# Autodesk Inventor assembly: spur_gear_m0.8-18.4
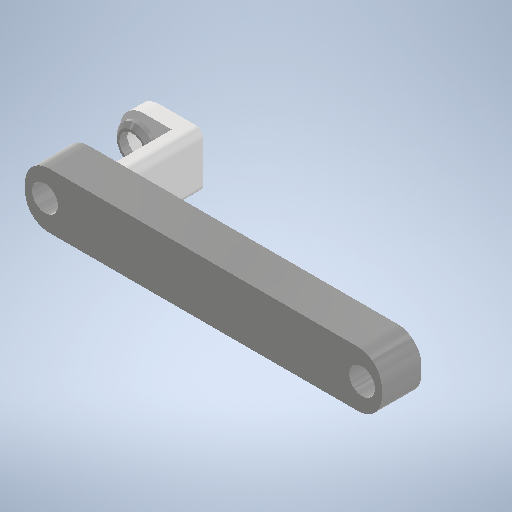
[picture p0: Inventor's stored thumbnail of the model, 512x512]
Saved by Autodesk Inventor 2025 (Build 290162000, 162)
## iProperties
Created: 2025-09-11
Part Number: spur_gear_m0.8-18.4
Document SubType Name: Assembly
Designer: sooo1
Author: sooo1
## Documents named in this file (4)
- C:\Users\sooo1\Documents\Inventor\MOBITOUCH\final\stroke_module_1\link_arm2_1.iam
- C:\Users\sooo1\Documents\Inventor\MOBITOUCH\final\stroke_module_1\link_arm1_2.iam
- C:\Users\sooo1\Documents\Inventor\MOBITOUCH\final\stroke_module_1\guide_link.ipt
- C:\Users\sooo1\Documents\Inventor\MOBITOUCH\final\stroke_module_1\spacer_Φ3.27_1.ipt
## Components (4 placed, 3 different names)
1. link_arm1_2:1 [sub-assembly] — メイト:1, フラッシュ:8, メイト:3, メイト:5, メイト:6, フラッシュ:10, メイト:7, メイト:8
2. guide_link:1 — メイト:5, メイト:6, フラッシュ:10, メイト:9, メイト:10
3. spacer_Φ3.27_1:1 — メイト:9, メイト:10
4. spacer_Φ3.27_1:2 — メイト:7, メイト:8
## Relationships (10: Mate 8, Flush 2)
- メイト:1 [Mate]: link_arm1_2:1
- フラッシュ:8 [Flush]: link_arm1_2:1
- メイト:3 [Mate]: link_arm1_2:1
- メイト:5 [Mate]: link_arm1_2:1 ↔ guide_link:1
- メイト:6 [Mate]: link_arm1_2:1 ↔ guide_link:1
- フラッシュ:10 [Flush]: link_arm1_2:1 ↔ guide_link:1
- メイト:7 [Mate]: link_arm1_2:1 ↔ spacer_Φ3.27_1:2
- メイト:8 [Mate]: link_arm1_2:1 ↔ spacer_Φ3.27_1:2
- メイト:9 [Mate]: guide_link:1 ↔ spacer_Φ3.27_1:1
- メイト:10 [Mate]: guide_link:1 ↔ spacer_Φ3.27_1:1
